# Autodesk Inventor assembly: assembly.rev5
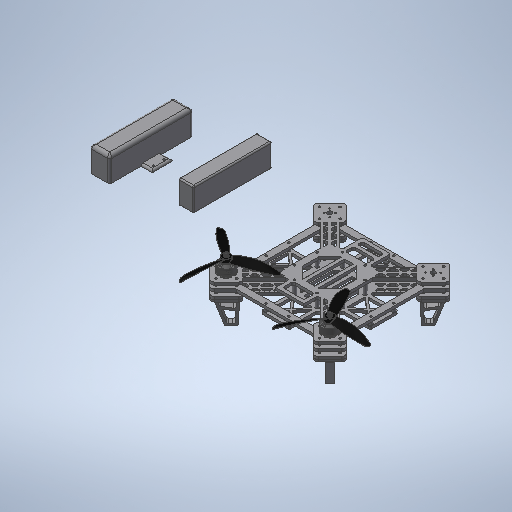
[picture p0: Inventor's stored thumbnail of the model, 512x512]
Saved by Autodesk Inventor 2025.2 (Build 292293000, 293)
## iProperties
Created: 2016-03-08
Part Number: assembly.rev5
Document SubType Name: Assembly
Designer: 200288284
Author: 200288284
## Documents named in this file (10)
- D:\UAV\机架\自制无人机 - 测试\assembly.rev5.iam
- D:\UAV\机架\自制无人机 - 测试\MOTOR_1806.iam
- D:\UAV\机架\自制无人机 - 测试\Tri-Blade 5045 Propeller\Tri-Blade 5045 Propeller\5045 CCW.ipt
- D:\UAV\机架\自制无人机 - 测试\电池.ipt
- D:\UAV\机架\自制无人机 - 测试\Tri-Blade 5045 Propeller\Protection_for_2.5_inch_prop.ipt
- D:\UAV\机架\自制无人机 - 测试\底板.ipt
- D:\UAV\机架\自制无人机 - 测试\中版.ipt
- D:\UAV\机架\自制无人机 - 测试\顶板.ipt
- D:\UAV\机架\自制无人机 - 测试\起落架一体.ipt
- D:\UAV\机架\自制无人机 - 测试\电池仓.ipt
## Components (15 placed, 9 different names)
1. 底板:1 — 配合:160, 配合:163, 配合:164, 配合:165, 配合:166, 配合:167, 配合:169, 配合:170, 配合:172, 配合:174, 配合:194, 配合:195, 配合:196, 配合:197, 配合:198, 配合:199
2. 中版:1 — 配合:160, 配合:161, 配合:162, 配合:194, 配合:195
3. 顶板:1 — 配合:161, 配合:162, 配合:163, 配合:178, 配合:179, 配合:180, 配合:181, 配合:182, 配合:184, 配合:185, 配合:187, 配合:192, 配合:193
4. 电池:2 — 配合:192
5. MOTOR_1806:5 [sub-assembly] — 配合:180, 配合:181, 配合:183, 配合:190, 配合:191
6. Protection_for_2.5_inch_prop:5 — 配合:182, 配合:183, 配合:184
7. 起落架一体:1 — 配合:164, 配合:174, 配合:196
8. 起落架一体:2 — 配合:166, 配合:172, 配合:198
9. 起落架一体:3 — 配合:165, 配合:170, 配合:199
10. 起落架一体:4 — 配合:167, 配合:169, 配合:197
11. MOTOR_1806:8 [sub-assembly] — 配合:178, 配合:179, 配合:186, 配合:188, 配合:189
12. Protection_for_2.5_inch_prop:6 — 配合:185, 配合:186, 配合:187
13. 5045 CCW:5 — 配合:188, 配合:189
14. 电池仓:1 — 配合:193
15. 5045 CCW:6 — 配合:190, 配合:191
## Relationships (34: Mate 34)
- 配合:160 [Mate]: 底板:1 ↔ 中版:1
- 配合:161 [Mate]: 中版:1 ↔ 顶板:1
- 配合:162 [Mate]: 中版:1 ↔ 顶板:1
- 配合:163 [Mate]: 底板:1 ↔ 顶板:1
- 配合:164 [Mate]: 底板:1 ↔ 起落架一体:1
- 配合:165 [Mate]: 底板:1 ↔ 起落架一体:3
- 配合:166 [Mate]: 底板:1 ↔ 起落架一体:2
- 配合:167 [Mate]: 底板:1 ↔ 起落架一体:4
- 配合:169 [Mate]: 底板:1 ↔ 起落架一体:4
- 配合:170 [Mate]: 底板:1 ↔ 起落架一体:3
- 配合:172 [Mate]: 底板:1 ↔ 起落架一体:2
- 配合:174 [Mate]: 底板:1 ↔ 起落架一体:1
- 配合:178 [Mate]: 顶板:1 ↔ MOTOR_1806:8
- 配合:179 [Mate]: 顶板:1 ↔ MOTOR_1806:8
- 配合:180 [Mate]: 顶板:1 ↔ MOTOR_1806:5
- 配合:181 [Mate]: 顶板:1 ↔ MOTOR_1806:5
- 配合:182 [Mate]: 顶板:1 ↔ Protection_for_2.5_inch_prop:5
- 配合:183 [Mate]: MOTOR_1806:5 ↔ Protection_for_2.5_inch_prop:5
- 配合:184 [Mate]: 顶板:1 ↔ Protection_for_2.5_inch_prop:5
- 配合:185 [Mate]: 顶板:1 ↔ Protection_for_2.5_inch_prop:6
- 配合:186 [Mate]: MOTOR_1806:8 ↔ Protection_for_2.5_inch_prop:6
- 配合:187 [Mate]: 顶板:1 ↔ Protection_for_2.5_inch_prop:6
- 配合:188 [Mate]: MOTOR_1806:8 ↔ 5045 CCW:5
- 配合:189 [Mate]: MOTOR_1806:8 ↔ 5045 CCW:5
- 配合:190 [Mate]: MOTOR_1806:5 ↔ 5045 CCW:6
- 配合:191 [Mate]: MOTOR_1806:5 ↔ 5045 CCW:6
- 配合:192 [Mate]: 顶板:1 ↔ 电池:2
- 配合:193 [Mate]: 顶板:1 ↔ 电池仓:1
- 配合:194 [Mate]: 底板:1 ↔ 中版:1
- 配合:195 [Mate]: 底板:1 ↔ 中版:1
- 配合:196 [Mate]: 底板:1 ↔ 起落架一体:1
- 配合:197 [Mate]: 底板:1 ↔ 起落架一体:4
- 配合:198 [Mate]: 底板:1 ↔ 起落架一体:2
- 配合:199 [Mate]: 底板:1 ↔ 起落架一体:3
